# Autodesk Inventor assembly: ASY MSC 100.1 roсket
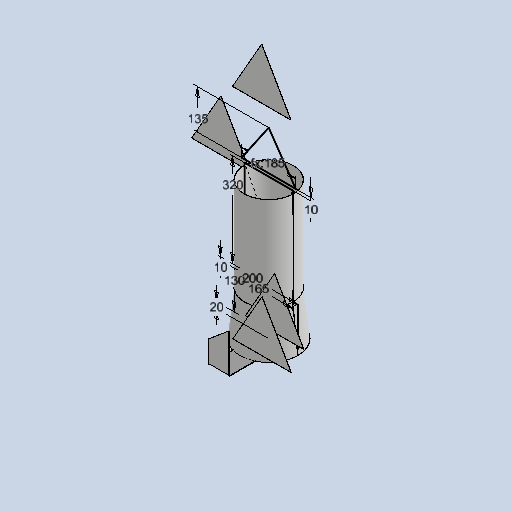
[picture p0: Inventor's stored thumbnail of the model, 512x512]
Saved by Autodesk Inventor 2025 (Build 290162010, 162A)
## iProperties
Created: 2024-05-19
Part Number: ASY MSC 100.1 roсket
Document SubType Name: Assembly
Designer: admin
Stock Number: ASY МОО 100.1 диффузор отбойник
Author: admin
## Documents named in this file (6)
- C:\Users\pokla\Documents\Inventor\Отстойник осветлитель\Manturovo_Se-clar-Gleb\ASY MSC 100.1 roсket.iam
- C:\Users\pokla\Documents\Inventor\Отстойник осветлитель\Manturovo_Se-clar-Gleb\MSC DIM 001 roсket sketch.ipt
- C:\Users\pokla\Documents\Inventor\Отстойник осветлитель\Manturovo_Se-clar-Gleb\MSC 101 roсket tail.ipt
- C:\Users\pokla\Documents\Inventor\Отстойник осветлитель\Manturovo_Se-clar-Gleb\MSC 102 roсket body.ipt
- C:\Users\pokla\Documents\Inventor\Отстойник осветлитель\Manturovo_Se-clar-Gleb\MSC 103 roсket nose.ipt
- C:\Users\pokla\Documents\Inventor\Отстойник осветлитель\Manturovo_Se-clar-Gleb\Part2.ipt
## Components (8 placed, 5 different names)
1. MSC DIM 001 roсket sketch:1
2. MSC 101 roсket tail:1 — Rigid:1, Mate:2
3. MSC 102 roсket body:1 — Rigid:1
4. MSC 103 roсket nose:1
5. MSC 103 roсket nose:2
6. MSC 103 roсket nose:3
7. MSC 103 roсket nose:4
8. Part2:1
## Relationships (2: WeldJoint 1, Mate 1)
- Rigid:1 [WeldJoint]: MSC 101 roсket tail:1 ↔ MSC 102 roсket body:1
- Mate:2: MSC 101 roсket tail:1
